# Autodesk Inventor assembly: Magnet Frame Straight for 4040 - Assembly
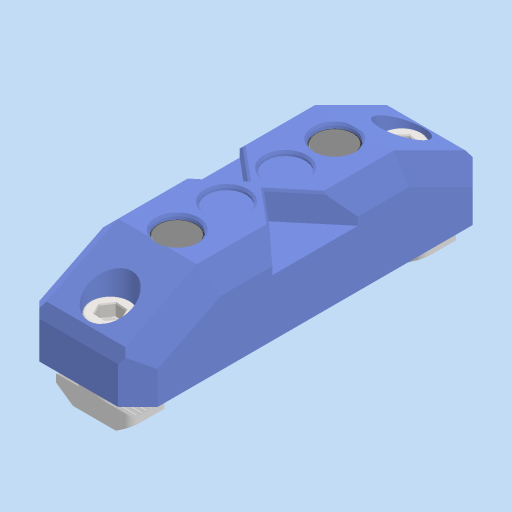
[picture p0: Inventor's stored thumbnail of the model, 512x512]
Saved by Autodesk Inventor 2023.2 (Build 272271000, 271)
## iProperties
Created: 2023-11-30
Part Number: Magnet Frame Straight for 4040 - Assembly
Document SubType Name: Assembly
Designer: Nils Bade
Author: Nils Bade
## Documents named in this file (5)
- C:\Users\nilsb\Documents\Inventor\Projektarbeit-Bade\Enclosure\Magnet Frame Straight for 4040 - Assembly.iam
- C:\Users\nilsb\Documents\Inventor\Projektarbeit-Bade\Enclosure\Magnet Frame straight for 4040.ipt
- C:\Users\nilsb\Documents\Inventor\Projektarbeit-Bade\Enclosure\Magnet-RatrigEnclosure.ipt
- C:\Users\nilsb\Documents\Inventor\Projektarbeit-Bade\Schrauben\Cap Head Screw M6x16.ipt
- C:\Users\nilsb\Documents\Inventor\Projektarbeit-Bade\RatRig_modified\T-NUT - DropIn 4040 SERIES - M6.ipt
## Components (7 placed, 4 different names)
1. Magnet Frame straight for 4040:1 — Passend:9, Passend:10, Passend:11, Passend:12, Passend:17, Passend:18, Passend:19, Passend:20
2. Cap Head Screw M6x16:1 — Passend:17, Passend:19
3. Cap Head Screw M6x16:2 — Passend:18, Passend:20
4. Magnet-RatrigEnclosure:1 — Passend:9, Passend:12
5. Magnet-RatrigEnclosure:2 — Passend:10, Passend:11
6. T-NUT - DROP IN TYPE FOR 40 SERIES - M6:1
7. T-NUT - DROP IN TYPE FOR 40 SERIES - M6:2
## Relationships (12: Mate 10, Angle 2)
- Passend:9 [Mate]: Magnet Frame straight for 4040:1 ↔ Magnet-RatrigEnclosure:1
- Passend:10 [Mate]: Magnet Frame straight for 4040:1 ↔ Magnet-RatrigEnclosure:2
- Passend:11 [Mate]: Magnet Frame straight for 4040:1 ↔ Magnet-RatrigEnclosure:2
- Passend:12 [Mate]: Magnet Frame straight for 4040:1 ↔ Magnet-RatrigEnclosure:1
- [Angle] (0 deg): Magnet Frame straight for 4040:1 ↔ T-NUT - DROP IN TYPE FOR 40 SERIES - M6:2
- [Angle] (0 deg): Magnet Frame straight for 4040:1 ↔ T-NUT - DROP IN TYPE FOR 40 SERIES - M6:1
- [Mate] (4.5 mm): Magnet Frame straight for 4040:1 ↔ T-NUT - DROP IN TYPE FOR 40 SERIES - M6:2
- [Mate] (4.5 mm): Magnet Frame straight for 4040:1 ↔ T-NUT - DROP IN TYPE FOR 40 SERIES - M6:1
- Passend:17 [Mate]: Magnet Frame straight for 4040:1 ↔ Cap Head Screw M6x16:1
- Passend:18 [Mate]: Magnet Frame straight for 4040:1 ↔ Cap Head Screw M6x16:2
- Passend:19 [Mate]: Magnet Frame straight for 4040:1 ↔ Cap Head Screw M6x16:1
- Passend:20 [Mate]: Magnet Frame straight for 4040:1 ↔ Cap Head Screw M6x16:2
